# Autodesk Inventor assembly: BD Drill Motor Mount assy 1
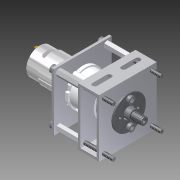
[picture p0: Inventor's stored thumbnail of the model, 180x180]
Saved by Autodesk Inventor 2012 (Build 160160000, 160)
## iProperties
Created: 2012-06-30
Part Number: BD Drill Motor Mount assy 1
Document SubType Name: Assembly
Designer: Bruce
Author: Bruce
## Documents named in this file (11)
- C:\Household Files\Bruce Work\Inventor Projects\2012 Drill motor Drives\BD Drill Motor Mount assy 1.iam
- C:\Household Files\Bruce Work\Inventor Projects\2012 Drill motor Drives\Slide Plate BD Motor mount.ipt
- C:\Household Files\Bruce Work\Inventor Projects\2012 Drill motor Drives\Btm Plate BD Motor mount.ipt
- C:\Household Files\Bruce Work\Inventor Projects\2012 Drill motor Drives\Top Plate BD Motor mount.ipt
- C:\Household Files\Bruce Work\Inventor Projects\2012 Drill motor Drives\Spring Ring BD drill motor mount.ipt
- C:\Household Files\Bruce Work\Inventor Projects\2012 Drill motor Drives\Stand offs BD motor mount.ipt
- C:\Household Files\Bruce Work\Inventor Projects\2012 Drill motor Drives\Bolt BD Drill motor mount.ipt
- C:\Household Files\Bruce Work\Inventor Projects\2012 Drill motor Drives\BD Drill motor assembly.iam
- C:\Household Files\Bruce Work\Inventor Projects\2012 Drill motor Drives\Spring BD drill motor.ipt
- C:\Household Files\Bruce Work\Inventor Projects\2012 Drill motor Drives\Spring torque cap.ipt
- C:\Household Files\Bruce Work\Inventor Projects\2012 Drill motor Drives\Bolt BD Drill motor spring.ipt
## Components (17 placed, 10 different names)
1. Slide Plate BD Motor mount:1 — Mate:1, Mate:2, Mate:3, Mate:6, Mate:7, Mate:25, Mate:26, Mate:27, Mate:28, Mate:31, Mate:32
2. Btm Plate BD Motor mount:1 — Mate:1, Mate:2, Mate:3, Mate:4, Mate:5, Mate:8, Mate:9, Mate:10, Mate:11, Mate:12, Mate:13, Mate:14, Mate:15
3. Top Plate BD Motor mount:1 — Mate:4, Mate:5, Mate:16, Mate:17, Mate:18, Mate:19, Mate:20, Mate:21, Mate:22, Mate:23, Mate:24
4. Spring Ring BD drill motor mount:1 — Mate:6, Mate:7, Mate:28, Mate:33, Mate:34
5. Stand offs BD motor mount:1 — Mate:8, Mate:14
6. Stand offs BD motor mount:2 — Mate:9, Mate:13, Mate:16
7. Stand offs BD motor mount:3 — Mate:10, Mate:12
8. Stand offs BD motor mount:4 — Mate:11, Mate:15
9. Bolt BD Drill motor mount:1 — Mate:17, Mate:21
10. Bolt BD Drill motor mount:2 — Mate:18, Mate:24
11. Bolt BD Drill motor mount:3 — Mate:20, Mate:23
12. Bolt BD Drill motor mount:4 — Mate:19, Mate:22
13. BD Drill motor assembly:1 [sub-assembly] — Mate:25, Mate:26, Mate:27, Mate:29, Mate:30, Angle:1
14. Spring BD drill motor:1 — Mate:29, Flush:1
15. Spring torque cap:1 — Mate:30, Flush:1, Angle:1
16. Bolt BD Drill motor spring:1 — Mate:31, Mate:33
17. Bolt BD Drill motor spring:2 — Mate:32, Mate:34
## Relationships (36: Mate 34, Flush 1, Angle 1)
- Mate:1: Slide Plate BD Motor mount:1 ↔ Btm Plate BD Motor mount:1
- Mate:2: Slide Plate BD Motor mount:1 ↔ Btm Plate BD Motor mount:1
- Mate:3: Slide Plate BD Motor mount:1 ↔ Btm Plate BD Motor mount:1
- Mate:4: Btm Plate BD Motor mount:1 ↔ Top Plate BD Motor mount:1
- Mate:5: Btm Plate BD Motor mount:1 ↔ Top Plate BD Motor mount:1
- Mate:6: Slide Plate BD Motor mount:1 ↔ Spring Ring BD drill motor mount:1
- Mate:7: Slide Plate BD Motor mount:1 ↔ Spring Ring BD drill motor mount:1
- Mate:8: Btm Plate BD Motor mount:1 ↔ Stand offs BD motor mount:1
- Mate:9: Btm Plate BD Motor mount:1 ↔ Stand offs BD motor mount:2
- Mate:10: Btm Plate BD Motor mount:1 ↔ Stand offs BD motor mount:3
- Mate:11: Btm Plate BD Motor mount:1 ↔ Stand offs BD motor mount:4
- Mate:12: Btm Plate BD Motor mount:1 ↔ Stand offs BD motor mount:3
- Mate:13: Btm Plate BD Motor mount:1 ↔ Stand offs BD motor mount:2
- Mate:14: Btm Plate BD Motor mount:1 ↔ Stand offs BD motor mount:1
- Mate:15: Btm Plate BD Motor mount:1 ↔ Stand offs BD motor mount:4
- Mate:16: Top Plate BD Motor mount:1 ↔ Stand offs BD motor mount:2
- Mate:17: Top Plate BD Motor mount:1 ↔ Bolt BD Drill motor mount:1
- Mate:18: Top Plate BD Motor mount:1 ↔ Bolt BD Drill motor mount:2
- Mate:19: Top Plate BD Motor mount:1 ↔ Bolt BD Drill motor mount:4
- Mate:20: Top Plate BD Motor mount:1 ↔ Bolt BD Drill motor mount:3
- Mate:21: Top Plate BD Motor mount:1 ↔ Bolt BD Drill motor mount:1
- Mate:22: Top Plate BD Motor mount:1 ↔ Bolt BD Drill motor mount:4
- Mate:23: Top Plate BD Motor mount:1 ↔ Bolt BD Drill motor mount:3
- Mate:24: Top Plate BD Motor mount:1 ↔ Bolt BD Drill motor mount:2
- Mate:25: Slide Plate BD Motor mount:1 ↔ BD Drill motor assembly:1
- Mate:26: Slide Plate BD Motor mount:1 ↔ BD Drill motor assembly:1
- Mate:27: Slide Plate BD Motor mount:1 ↔ BD Drill motor assembly:1
- Mate:28: Slide Plate BD Motor mount:1 ↔ Spring Ring BD drill motor mount:1
- Mate:29: BD Drill motor assembly:1 ↔ Spring BD drill motor:1
- Mate:30: BD Drill motor assembly:1 ↔ Spring torque cap:1
- Flush:1 (1.27 mm): Spring BD drill motor:1 ↔ Spring torque cap:1
- Angle:1 (0 deg): BD Drill motor assembly:1 ↔ Spring torque cap:1
- Mate:31: Slide Plate BD Motor mount:1 ↔ Bolt BD Drill motor spring:1
- Mate:32: Slide Plate BD Motor mount:1 ↔ Bolt BD Drill motor spring:2
- Mate:33: Spring Ring BD drill motor mount:1 ↔ Bolt BD Drill motor spring:1
- Mate:34: Spring Ring BD drill motor mount:1 ↔ Bolt BD Drill motor spring:2
